# Autodesk Inventor assembly: napinacz_zlozenie
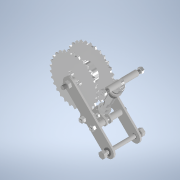
[picture p0: Inventor's stored thumbnail of the model, 180x180]
Saved by Autodesk Inventor 2020.3 (Build 243373000, 373)
## iProperties
Created: 2021-11-03
Part Number: napinacz_zlozenie
Document SubType Name: Assembly
Designer: patry
Author: patry
## Documents named in this file (20)
- C:\Users\patry\Desktop\Semestr 7\Inzynierka\Projekt inventor\Ariadna_inzynierka\Workspaces\Obszar roboczy\Obszar roboczy\Naped\Zawieszenie_v3\napinacz_zlozenie.iam
- C:\Users\patry\Desktop\Semestr 7\Inzynierka\Projekt inventor\Ariadna_inzynierka\Workspaces\Obszar roboczy\Obszar roboczy\Naped\Kola\kolo_przednie.iam
- C:\Users\patry\Desktop\Semestr 7\Inzynierka\Projekt inventor\Ariadna_inzynierka\Workspaces\Obszar roboczy\Obszar roboczy\Naped\Zawieszenie_v3\ramie_napinacza.ipt
- C:\Users\patry\Desktop\Semestr 7\Inzynierka\Projekt inventor\Ariadna_inzynierka\Workspaces\Obszar roboczy\Obszar roboczy\Naped\Amortyzator\Korpus.ipt
- C:\Users\patry\Desktop\Semestr 7\Inzynierka\Projekt inventor\Ariadna_inzynierka\Workspaces\Obszar roboczy\Obszar roboczy\Naped\Amortyzator\Tlok.ipt
- C:\Users\patry\Desktop\Semestr 7\Inzynierka\Projekt inventor\Ariadna_inzynierka\Workspaces\Obszar roboczy\Obszar roboczy\Naped\Amortyzator\Nakretka.ipt
- C:\Users\patry\Desktop\Semestr 7\Inzynierka\Projekt inventor\Ariadna_inzynierka\Workspaces\Obszar roboczy\Obszar roboczy\Naped\Sruby\M5_nut_5mm.ipt
- C:\Users\patry\Desktop\Semestr 7\Inzynierka\Projekt inventor\Ariadna_inzynierka\Workspaces\Obszar roboczy\Obszar roboczy\Naped\Sruby\M5_70_shaft.ipt
- C:\Users\patry\Desktop\Semestr 7\Inzynierka\Projekt inventor\Ariadna_inzynierka\Workspaces\Obszar roboczy\Obszar roboczy\Naped\Sruby\M3_16_shaft.ipt
- C:\Users\patry\Desktop\Semestr 7\Inzynierka\Projekt inventor\Ariadna_inzynierka\Workspaces\Obszar roboczy\Obszar roboczy\Naped\Sruby\M3_nut_2,5mm.ipt
- C:\Users\patry\Desktop\Semestr 7\Inzynierka\Projekt inventor\Ariadna_inzynierka\Workspaces\Obszar roboczy\Obszar roboczy\Naped\Zawieszenie_v3\wspornik_amortyzatora.ipt
- C:\Users\patry\Desktop\Semestr 7\Inzynierka\Projekt inventor\Ariadna_inzynierka\Workspaces\Obszar roboczy\Obszar roboczy\Naped\Sruby\tuleja_M5_M9_20.ipt
- C:\Users\patry\Desktop\Semestr 7\Inzynierka\Projekt inventor\Ariadna_inzynierka\Workspaces\Obszar roboczy\Obszar roboczy\Naped\Sruby\tuleja_M5_M9_25.ipt
- C:\Users\patry\Desktop\Semestr 7\Inzynierka\Projekt inventor\Ariadna_inzynierka\Workspaces\Obszar roboczy\Obszar roboczy\Naped\Sruby\M5_60_shaft.ipt
- C:\Users\patry\Desktop\Semestr 7\Inzynierka\Projekt inventor\Ariadna_inzynierka\Workspaces\Obszar roboczy\Obszar roboczy\Naped\Zawieszenie_v3\tuleja_TUF106040.ipt
- C:\Users\patry\Desktop\Semestr 7\Inzynierka\Projekt inventor\Ariadna_inzynierka\Workspaces\Obszar roboczy\Obszar roboczy\Naped\Sruby\M6_70_shaft.ipt
- C:\Users\patry\Desktop\Semestr 7\Inzynierka\Projekt inventor\Ariadna_inzynierka\Workspaces\Obszar roboczy\Obszar roboczy\Naped\Sruby\M6_nut_5mm.ipt
- C:\Users\patry\Desktop\Semestr 7\Inzynierka\Projekt inventor\Ariadna_inzynierka\Workspaces\Obszar roboczy\Obszar roboczy\Naped\Sruby\tuleja_M5_M9_13.ipt
- C:\Users\patry\Desktop\Semestr 7\Inzynierka\Projekt inventor\Ariadna_inzynierka\Workspaces\Obszar roboczy\Obszar roboczy\Naped\Sruby\tuleja_M5_M9_18.ipt
- C:\Users\patry\Desktop\Semestr 7\Inzynierka\Projekt inventor\Ariadna_inzynierka\Workspaces\Obszar roboczy\Obszar roboczy\Naped\Sruby\tuleja_M6_M10_8.ipt
## Components (34 placed, 19 different names)
1. kolo_przednie:1 [sub-assembly] — Zestawiające:57, Zestawiające:58
2. ramie_napinacza:1 — Zestawiające:49, Zestawiające:50, Zestawiające:51, Zestawiające:52, Zestawiające:53, Zestawiające:57, Zestawiające:58, Zestawiające:59, Równoległe:4, Zestawiające:60, Równoległe:5, Zestawiające:64, Zestawiające:70, Zestawiające:74, Zestawiające:75, Równoległe:7, Zestawiające:77, Zestawiające:81
3. Korpus:1
4. Tlok:1
5. Nakretka:1
6. M5_nut_5mm:1 — Równoległe:6
7. M5_70_shaft:1
8. M5_nut_5mm:2
9. M3_16_shaft:1
10. M3_nut_2,5mm:1
11. M3_nut_2,5mm:2
12. wspornik_amortyzatora:1 — Zestawiające:62, Zestawiające:63
13. wspornik_amortyzatora:2 — Zestawiające:72
14. M5_nut_5mm:3 — Zestawiające:69, Zestawiające:70
15. M5_nut_5mm:4 — Zestawiające:61, Zestawiające:64
16. M5_nut_5mm:5 — Zestawiające:65, Zestawiające:66
17. M5_nut_5mm:6 — Zestawiające:67, Zestawiające:68
18. tuleja_M5_M9_20:1
19. tuleja_M5_M9_25:1
20. ramie_napinacza:2 — Zestawiające:49, Zestawiające:50, Zestawiające:51, Zestawiające:54, Zestawiające:55, Równoległe:3, Zestawiające:66, Zestawiające:68, Zestawiające:79, Zestawiające:83
21. M5_60_shaft:1 — Zestawiające:59, Równoległe:4, Zestawiające:61, Zestawiające:62, Zestawiające:65, Zestawiające:71, Zestawiające:73
22. M5_60_shaft:2 — Zestawiające:60, Równoległe:5, Zestawiające:63, Zestawiające:67, Zestawiające:69
23. tuleja_TUF106040:1 — Zestawiające:52, Zestawiające:53, Zestawiające:56
24. tuleja_TUF106040:2 — Zestawiające:54, Zestawiające:55
25. M6_70_shaft:1 — Równoległe:3
26. M6_nut_5mm:1 — Zestawiające:56
27. M6_nut_5mm:2 — Równoległe:6
28. tuleja_M5_M9_13:1 — Zestawiające:73, Zestawiające:74
29. tuleja_M5_M9_18:1 — Zestawiające:71, Zestawiające:72
30. M6_70_shaft:2 — Zestawiające:75, Równoległe:7, Zestawiające:76, Zestawiające:78, Zestawiające:80, Zestawiające:82
31. M6_nut_5mm:3 — Zestawiające:76, Zestawiające:77
32. M6_nut_5mm:4 — Zestawiające:78, Zestawiające:79
33. tuleja_M6_M10_8:1 — Zestawiające:80, Zestawiające:81
34. tuleja_M6_M10_8:2 — Zestawiające:82, Zestawiające:83
## Relationships (70: Mate 61, Flush 7, Angle 1, CylindricalJoint 1)
- [Mate]: Korpus:1 ↔ Tlok:1
- [Angle] (0 deg): Korpus:1 ↔ Tlok:1
- [Mate]: Korpus:1 ↔ Nakretka:1
- [Mate] (5 mm): Korpus:1 ↔ Nakretka:1
- [CylindricalJoint]: Korpus:1 ↔ Tlok:1
- [Mate]: Korpus:1 ↔ M5_70_shaft:1
- [Flush] (-30 mm): Korpus:1 ↔ M5_70_shaft:1
- [Mate]: M5_nut_5mm:1 ↔ M5_70_shaft:1
- [Mate]: M5_70_shaft:1 ↔ M5_nut_5mm:2
- [Mate] (60 mm): M5_nut_5mm:1 ↔ M5_nut_5mm:2
- [Mate] (30 mm): Korpus:1 ↔ M5_nut_5mm:1
- [Mate]: wspornik_amortyzatora:1 ↔ wspornik_amortyzatora:2
- [Mate]: wspornik_amortyzatora:1 ↔ wspornik_amortyzatora:2
- [Mate] (5 mm): wspornik_amortyzatora:1 ↔ wspornik_amortyzatora:2
- [Mate]: M3_16_shaft:1 ↔ wspornik_amortyzatora:2
- [Flush] (-2.5 mm): M3_16_shaft:1 ↔ wspornik_amortyzatora:1
- [Mate]: M3_16_shaft:1 ↔ M3_nut_2,5mm:1
- [Mate]: M3_nut_2,5mm:1 ↔ wspornik_amortyzatora:1
- [Mate]: M3_16_shaft:1 ↔ M3_nut_2,5mm:2
- [Mate]: M3_nut_2,5mm:2 ↔ wspornik_amortyzatora:2
- [Mate]: Tlok:1 ↔ M3_16_shaft:1
- [Mate]: Tlok:1 ↔ wspornik_amortyzatora:2
- [Mate]: M5_70_shaft:1 ↔ tuleja_M5_M9_20:1
- [Mate]: Korpus:1 ↔ tuleja_M5_M9_20:1
- [Mate]: M5_70_shaft:1 ↔ tuleja_M5_M9_25:1
- [Mate]: Korpus:1 ↔ tuleja_M5_M9_25:1
- [Mate]: M6_70_shaft:1 ↔ M6_nut_5mm:1
- [Mate]: M6_70_shaft:1 ↔ M6_nut_5mm:2
- [Mate] (60 mm): M6_nut_5mm:1 ↔ M6_nut_5mm:2
- [Mate]: tuleja_TUF106040:1 ↔ M6_70_shaft:1
- Zestawiające:49 [Mate]: ramie_napinacza:1 ↔ ramie_napinacza:2
- Zestawiające:50 [Mate]: ramie_napinacza:1 ↔ ramie_napinacza:2
- Zestawiające:51 [Mate] (42 mm): ramie_napinacza:1 ↔ ramie_napinacza:2
- Zestawiające:52 [Mate]: ramie_napinacza:1 ↔ tuleja_TUF106040:1
- Zestawiające:53 [Mate]: ramie_napinacza:1 ↔ tuleja_TUF106040:1
- Zestawiające:54 [Mate]: ramie_napinacza:2 ↔ tuleja_TUF106040:2
- Zestawiające:55 [Mate]: ramie_napinacza:2 ↔ tuleja_TUF106040:2
- Zestawiające:56 [Mate] (5 mm): tuleja_TUF106040:1 ↔ M6_nut_5mm:1
- Równoległe:3 [Flush] (-11 mm): ramie_napinacza:2 ↔ M6_70_shaft:1
- Zestawiające:57 [Mate] (5.5 mm): kolo_przednie:1 ↔ ramie_napinacza:1
- Zestawiające:58 [Mate]: kolo_przednie:1 ↔ ramie_napinacza:1
- Zestawiające:59 [Mate]: ramie_napinacza:1 ↔ M5_60_shaft:1
- Równoległe:4 [Flush] (6 mm): ramie_napinacza:1 ↔ M5_60_shaft:1
- Zestawiające:60 [Mate]: ramie_napinacza:1 ↔ M5_60_shaft:2
- Równoległe:5 [Flush] (6 mm): ramie_napinacza:1 ↔ M5_60_shaft:2
- Zestawiające:61 [Mate]: M5_nut_5mm:4 ↔ M5_60_shaft:1
- Zestawiające:62 [Mate]: wspornik_amortyzatora:1 ↔ M5_60_shaft:1
- Zestawiające:63 [Mate]: wspornik_amortyzatora:1 ↔ M5_60_shaft:2
- Zestawiające:64 [Mate]: ramie_napinacza:1 ↔ M5_nut_5mm:4
- Zestawiające:65 [Mate]: M5_nut_5mm:5 ↔ M5_60_shaft:1
- Zestawiające:66 [Mate]: M5_nut_5mm:5 ↔ ramie_napinacza:2
- Zestawiające:67 [Mate]: M5_nut_5mm:6 ↔ M5_60_shaft:2
- Zestawiające:68 [Mate]: M5_nut_5mm:6 ↔ ramie_napinacza:2
- Zestawiające:69 [Mate]: M5_nut_5mm:3 ↔ M5_60_shaft:2
- Zestawiające:70 [Mate]: ramie_napinacza:1 ↔ M5_nut_5mm:3
- Równoległe:6 [Flush]: M5_nut_5mm:1 ↔ M6_nut_5mm:2
- Zestawiające:71 [Mate]: M5_60_shaft:1 ↔ tuleja_M5_M9_18:1
- Zestawiające:72 [Mate]: wspornik_amortyzatora:2 ↔ tuleja_M5_M9_18:1
- Zestawiające:73 [Mate]: M5_60_shaft:1 ↔ tuleja_M5_M9_13:1
- Zestawiające:74 [Mate]: ramie_napinacza:1 ↔ tuleja_M5_M9_13:1
- Zestawiające:75 [Mate]: ramie_napinacza:1 ↔ M6_70_shaft:2
- Równoległe:7 [Flush] (-11 mm): ramie_napinacza:1 ↔ M6_70_shaft:2
- Zestawiające:76 [Mate]: M6_70_shaft:2 ↔ M6_nut_5mm:3
- Zestawiające:77 [Mate]: ramie_napinacza:1 ↔ M6_nut_5mm:3
- Zestawiające:78 [Mate]: M6_70_shaft:2 ↔ M6_nut_5mm:4
- Zestawiające:79 [Mate]: ramie_napinacza:2 ↔ M6_nut_5mm:4
- Zestawiające:80 [Mate]: M6_70_shaft:2 ↔ tuleja_M6_M10_8:1
- Zestawiające:81 [Mate]: ramie_napinacza:1 ↔ tuleja_M6_M10_8:1
- Zestawiające:82 [Mate]: M6_70_shaft:2 ↔ tuleja_M6_M10_8:2
- Zestawiające:83 [Mate]: ramie_napinacza:2 ↔ tuleja_M6_M10_8:2
## Named parameters: d83_d6 = -2 mm, d84_d7 = -12.94136 mm, d85_d8 = -13 mm, d86_d0 = 0 mm, d87_d1 = 0 deg, d88_d3 = 0 mm, d89_d4 = 5 mm, d90_d5 = 0 deg
